# Autodesk Inventor assembly: workbench
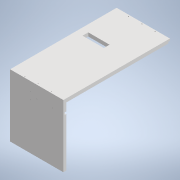
[picture p0: Inventor's stored thumbnail of the model, 180x180]
Saved by Autodesk Inventor 2022 (Build 260153000, 153)
## iProperties
Created: 2022-02-20
Part Number: workbench
Document SubType Name: Assembly
Designer: MarkP
Author: MarkP
## Documents named in this file (3)
- C:\Users\MarkP\Documents\Mark\workbench.iam
- C:\Users\MarkP\Documents\Mark\bench.ipt
- C:\Users\MarkP\Documents\Mark\wall.ipt
## Components (2 placed, 2 different names)
1. bench:1 — Mate:1, Mate:2, Flush:1
2. wall:1 — Mate:1, Mate:2, Flush:1
## Relationships (3: Mate 2, Flush 1)
- Mate:1: bench:1 ↔ wall:1
- Mate:2: bench:1 ↔ wall:1
- Flush:1: bench:1 ↔ wall:1
